# Autodesk Inventor assembly: rail_mount
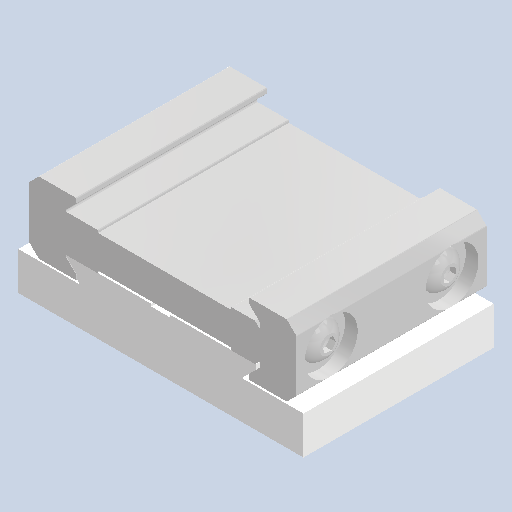
[picture p0: Inventor's stored thumbnail of the model, 512x512]
Saved by Autodesk Inventor 2026.1 (Build 301233000, 233)
## iProperties
Created: 2019-05-24
Part Number: rail_mount
Document SubType Name: Assembly
Designer: Julian
Author: Julian
## Documents named in this file (3)
- C:\Users\user\Desktop\setup for publishing\rail_mount.iam
- C:\Users\user\Desktop\setup for publishing\XT66C2-Step_rail mount.ipt
- C:\Users\user\Desktop\setup for publishing\XT66D2-40-Step_post_mount.ipt
## Components (2 placed, 2 different names)
1. XT66C2-Step_rail mount:1 — Mate:5, Mate:6, Flush:1
2. XT66D2-40-Step_post_mount:1 — Mate:5, Mate:6, Flush:1
## Relationships (3: Mate 2, Flush 1)
- Mate:5: XT66C2-Step_rail mount:1 ↔ XT66D2-40-Step_post_mount:1
- Mate:6: XT66C2-Step_rail mount:1 ↔ XT66D2-40-Step_post_mount:1
- Flush:1 (-0.0508 mm): XT66C2-Step_rail mount:1 ↔ XT66D2-40-Step_post_mount:1
